# Autodesk Inventor assembly: estanteria
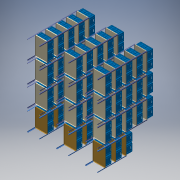
[picture p0: Inventor's stored thumbnail of the model, 180x180]
Saved by Autodesk Inventor 2016 (Build 200138000, 138)
## iProperties
Created: 2015-11-23
Part Number: estanteria
Material: Genérico
Document SubType Name: Assembly
Designer: David
Author: David
## Documents named in this file (4)
- D:\Programas\xampp\htdocs\localUnal\storage\macros\cuarto\Modelado\estanteria.iam
- D:\Programas\xampp\htdocs\localUnal\storage\macros\cuarto\Modelado\estantería\Estante Pequeño\Estante Pequeño.iam
- D:\Programas\xampp\htdocs\localUnal\storage\macros\cuarto\Modelado\estantería\Estantes Grandes\Estante.iam
- D:\Programas\xampp\htdocs\localUnal\storage\macros\cuarto\Modelado\Puente inventor.xlsx
## Components (54 placed, 2 different names)
1. Estante Pequeño:1 [sub-assembly] — Nivelación:1, Nivelación:2, Coincidencia:1
2. Estante Pequeño:2 [sub-assembly]
3. Estante Pequeño:3 [sub-assembly]
4. Estante Pequeño:4 [sub-assembly]
5. Estante Pequeño:5 [sub-assembly]
6. Estante Pequeño:6 [sub-assembly]
7. Estante:1 [sub-assembly] — Nivelación:1, Nivelación:2, Coincidencia:1
8. Estante:2 [sub-assembly]
9. Estante:3 [sub-assembly]
10. Estante:4 [sub-assembly]
11. Estante:5 [sub-assembly]
12. Estante:6 [sub-assembly]
13. Estante:7 [sub-assembly]
14. Estante:8 [sub-assembly]
15. Estante:9 [sub-assembly]
16. Estante:10 [sub-assembly]
17. Estante:11 [sub-assembly]
18. Estante:12 [sub-assembly]
19. Estante:13 [sub-assembly]
20. Estante:14 [sub-assembly]
21. Estante:15 [sub-assembly]
22. Estante:16 [sub-assembly]
23. Estante:17 [sub-assembly]
24. Estante:18 [sub-assembly]
25. Estante:19 [sub-assembly]
26. Estante:20 [sub-assembly]
27. Estante:21 [sub-assembly]
28. Estante:22 [sub-assembly]
29. Estante:23 [sub-assembly]
30. Estante:24 [sub-assembly]
31. Estante:25 [sub-assembly]
32. Estante:26 [sub-assembly]
33. Estante:27 [sub-assembly]
34. Estante:28 [sub-assembly]
35. Estante:29 [sub-assembly]
36. Estante:30 [sub-assembly]
37. Estante:31 [sub-assembly]
38. Estante:32 [sub-assembly]
39. Estante:33 [sub-assembly]
40. Estante:34 [sub-assembly]
41. Estante:35 [sub-assembly]
42. Estante:36 [sub-assembly]
43. Estante:37 [sub-assembly]
44. Estante:38 [sub-assembly]
45. Estante:39 [sub-assembly]
46. Estante:40 [sub-assembly]
47. Estante:41 [sub-assembly]
48. Estante:42 [sub-assembly]
49. Estante:43 [sub-assembly]
50. Estante:44 [sub-assembly]
51. Estante:45 [sub-assembly]
52. Estante:46 [sub-assembly]
53. Estante:47 [sub-assembly]
54. Estante:48 [sub-assembly]
## Component patterns: (6 elements, first: Estante Pequeño:1), (48 elements, first: Estante:1)
## Relationships (3: Flush 2, Mate 1)
- Nivelación:1 [Flush]: Estante Pequeño:1 ↔ Estante:1
- Nivelación:2 [Flush]: Estante Pequeño:1 ↔ Estante:1
- Coincidencia:1 [Mate] (100 mm): Estante Pequeño:1 ↔ Estante:1
## Named parameters: PL_N = 10000 mm, PA_N = 3500 mm, PE_N = 50.8 mm, PL_S = 10000 mm, PA_S = 3500 mm, PE_S = 50.8 mm, DP_S = 5750 mm, AP_S = 2000 mm, PL_EO = 10000 mm, PA_EO = 3500 mm, PE_EO = 50.8 mm, T_L = 10000 mm, T_A = 10000 mm, T_E = 50.8 mm, lon_ve = 320 mm, n_a = 3 mm, t_a = 19.05 mm, d_a = 80 mm, lon_ho = 550 mm, d_bor = 44 mm, lon_gui = 137.5 mm, esp_gui = 288 mm, lon_ve2 = 498.475 mm, n_a2 = 3 mm, t_a2 = 124.61875 mm, d_a2 = 124.61875 mm, lon_ho2 = 933.45 mm, d_bor2 = 74.676 mm, lon_gui2 = 233.3625 mm, esp_gui2 = 448.6275 mm, UE_L = 3130 mm, UE_A = 640 mm, UE_AN = 550 mm, UC_L = 1314.45 mm, UC_A = 996.95 mm, UC_AN = 933.45 mm, A_ET = 35 mm, E_EP = 20 mm, SEP_NS = 0 mm, SEP_EW = 1400 mm, CEP_NS = 1, CEP_EW = 6, DSEG = 0 mm, AEGEP_NS = 0 mm, SEPEG_NS = 100 mm, SEG_NS = 1000 mm, SEG_EW = 1400 mm, CEG_NS = 8, CEG_EW = 6, DNS = 550 mm, DEW = 1200 mm
